# Autodesk Inventor assembly: CarAssembly mk4
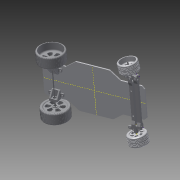
[picture p0: Inventor's stored thumbnail of the model, 180x180]
Saved by Autodesk Inventor 2015 (Build 190159000, 159)
## iProperties
Created: 2014-11-06
Part Number: CarAssembly mk4
Document SubType Name: Assembly
Designer: ah14592
Author: ah14592
## Documents named in this file (10)
- \\ads.bris.ac.uk\filestore\MyFiles\StudentPG1\ah14592\Documents\Inventor\Assembly\CarAssembly mk4.iam
- \\ads.bris.ac.uk\filestore\MyFiles\StudentPG1\ah14592\Documents\Inventor\Steering\Steering T\Part3.ipt
- \\ads.bris.ac.uk\filestore\MyFiles\StudentPG1\ah14592\Documents\Inventor\Steering\T Connector Rod\Part1.ipt
- \\ads.bris.ac.uk\filestore\MyFiles\StudentPG1\ah14592\Documents\Inventor\Wheels\Front Wheels\Wheels1.ipt
- \\ads.bris.ac.uk\filestore\MyFiles\StudentPG1\ah14592\Documents\Inventor\Front connectors.ipt
- \\ads.bris.ac.uk\filestore\MyFiles\StudentPG1\ah14592\Documents\Inventor\Base\Basetrimed.ipt
- \\ads.bris.ac.uk\filestore\MyFiles\StudentPG1\ah14592\Documents\Inventor\Rear Axel Holder\holder1_MIR1.ipt
- \\ads.bris.ac.uk\filestore\MyFiles\StudentPG1\ah14592\Documents\Inventor\RearAxel.ipt
- \\ads.bris.ac.uk\filestore\MyFiles\StudentPG1\ah14592\Documents\Inventor\Wheels\Rear Wheels\Wheels1.ipt
- \\ads.bris.ac.uk\filestore\MyFiles\StudentPG1\ah14592\Documents\Inventor\Steering\Steering Rod\mk4.ipt
## Components (14 placed, 8 different names)
1. Part3:1 — Mate:28, Mate:29
2. Part3:2 — Mate:21, Mate:22, Mate:30
3. Part1:1
4. Front connectors:1
5. Basetrimed:1
6. holder1_MIR1:1
7. holder1_MIR1:2
8. RearAxel:1
9. Wheels1:1
10. Wheels1:2 — Mate:23, Flush:11
11. Wheels1:3
12. Wheels1:4
13. Front connectors:2 — Mate:21, Mate:22, Mate:23, Flush:11
14. mk4:2 — Mate:28, Mate:29, Mate:30
## Relationships (31: Mate 20, Flush 11)
- [Mate]: Part3:1 ↔ Part1:1
- [Mate]: Part3:1 ↔ Part1:1
- [Mate]: Part3:2 ↔ Part1:1
- [Mate]: Part3:2 ↔ Part1:1
- [Mate]: Part3:1 ↔ Front connectors:1
- [Mate]: Part3:1 ↔ Front connectors:1
- [Mate]: Front connectors:1 ↔ Wheels1:1
- [Flush] (15 mm): Front connectors:1 ↔ Wheels1:1
- [Mate]: Part1:1 ↔ Basetrimed:1
- [Flush] (30 mm): Part1:1 ↔ Basetrimed:1
- [Mate]: Basetrimed:1 ↔ holder1_MIR1:1
- [Mate]: Basetrimed:1 ↔ holder1_MIR1:2
- [Flush]: Basetrimed:1 ↔ holder1_MIR1:1
- [Flush]: Basetrimed:1 ↔ holder1_MIR1:2
- [Flush] (15 mm): Basetrimed:1 ↔ holder1_MIR1:2
- [Flush] (15 mm): Basetrimed:1 ↔ holder1_MIR1:1
- [Mate]: holder1_MIR1:2 ↔ RearAxel:1
- [Mate]: holder1_MIR1:1 ↔ RearAxel:1
- [Flush] (29 mm): holder1_MIR1:1 ↔ RearAxel:1
- [Mate]: RearAxel:1 ↔ Wheels1:4
- [Mate]: RearAxel:1 ↔ Wheels1:3
- [Flush] (5 mm): RearAxel:1 ↔ Wheels1:3
- [Flush] (5 mm): RearAxel:1 ↔ Wheels1:4
- [Flush] (28 mm): Part1:1 ↔ Basetrimed:1
- Mate:21: Part3:2 ↔ Front connectors:2
- Mate:22: Part3:2 ↔ Front connectors:2
- Mate:23: Wheels1:2 ↔ Front connectors:2
- Flush:11 (15 mm): Wheels1:2 ↔ Front connectors:2
- Mate:28: Part3:1 ↔ mk4:2
- Mate:29: Part3:1 ↔ mk4:2
- Mate:30: Part3:2 ↔ mk4:2
## Named parameters: d16_d28 = 0 mm, d17_d29 = 0 mm
